# Autodesk Inventor assembly: Robot
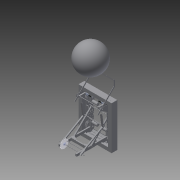
[picture p0: Inventor's stored thumbnail of the model, 180x180]
Saved by Autodesk Inventor 2013 (Build 170138000, 138)
## iProperties
Created: 2014-01-18
Part Number: Robot
Document SubType Name: Assembly
Designer: 272817
Author: 272817
## Documents named in this file (8)
- E:\Robotics\FRC\2014\CAD\Robot\Robot.iam
- E:\Robotics\FRC\2014\CAD\Robot\Frame\Robot Chassis 2014.iam
- E:\Robotics\FRC\2014\CAD\Robot\Bumpers\Bumpers.iam
- E:\Robotics\FRC\2014\CAD\Robot\Catapult\Catapult.iam
- E:\Robotics\FRC\2014\CAD\Brian's Derp\Additions\Ball.ipt
- E:\Robotics\FRC\2014\CAD\Robot\Catapult\Arm\ArmSquare.iam
- E:\Robotics\FRC\2014\CAD\Robot\Pickup\Structure.iam
- E:\Robotics\FRC\2014\CAD\Robot\Pickup\Arms.iam
## Components (7 placed, 7 different names)
1. Robot Chassis 2014:1 [sub-assembly] — Mate:1, Mate:2, Flush:1, Mate:4, Mate:5, Mate:6, Mate:14, Flush:2
2. Bumpers:1 [sub-assembly] — Mate:1, Mate:2, Flush:1, Mate:13
3. Catapult:1 [sub-assembly] — Mate:4, Mate:5, Mate:6, Mate:10, Mate:11, Mate:12
4. Ball:1 — Mate:10
5. ArmSquare:2 [sub-assembly] — Mate:11, Mate:12
6. Structure:1 [sub-assembly] — Mate:13, Mate:14, Flush:2, Mate:15, Mate:16
7. Arms:1 [sub-assembly] — Mate:15, Mate:16
## Relationships (14: Mate 12, Flush 2)
- Mate:1: Robot Chassis 2014:1 ↔ Bumpers:1
- Mate:2 (0.127 mm): Robot Chassis 2014:1 ↔ Bumpers:1
- Flush:1 (30.1625 mm): Robot Chassis 2014:1 ↔ Bumpers:1
- Mate:4: Robot Chassis 2014:1 ↔ Catapult:1
- Mate:5: Robot Chassis 2014:1 ↔ Catapult:1
- Mate:6 (-12.7 mm): Robot Chassis 2014:1 ↔ Catapult:1
- Mate:10 (177.8 mm): Catapult:1 ↔ Ball:1
- Mate:11 (3.175 mm): Catapult:1 ↔ ArmSquare:2
- Mate:12: Catapult:1 ↔ ArmSquare:2
- Mate:13: Bumpers:1 ↔ Structure:1
- Mate:14: Robot Chassis 2014:1 ↔ Structure:1
- Flush:2: Robot Chassis 2014:1 ↔ Structure:1
- Mate:15: Structure:1 ↔ Arms:1
- Mate:16: Structure:1 ↔ Arms:1
